# Autodesk Inventor assembly: Wall Cabinet 2 Door
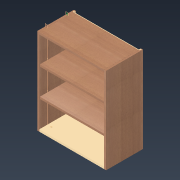
[picture p0: Inventor's stored thumbnail of the model, 180x180]
Saved by Autodesk Inventor 2022 (Build 260153000, 153)
## iProperties
Created: 2017-01-25
Part Number: Wall Cabinet 2 Door
Document SubType Name: Assembly
Designer: SvetlanaB
Author: SvetlanaB
## iProperties of the stored document MemberDocs/xAaaaqbcaAaaaaaaaAaaaqxjcCb
Created: 2017-01-25
Part Number: Wall Cabinet 2 Door
Document SubType Name: Assembly
Designer: SvetlanaB
Author: SvetlanaB
## Documents named in this file (26)
- C:\W4INV 2024 Design\iBOX LIBRARY\Kitchen\Wall Cabinets\Wall cabinet\Wall Cabinet.iam
- C:\W4INV 2022 Design\iBOX LIBRARY\Kitchen\Wall Cabinets\Wall cabinet\Right panel.ipt
- C:\W4INV 2022 Design\iBOX LIBRARY\Kitchen\Wall Cabinets\Wall cabinet\Top panel.ipt
- C:\W4INV 2022 Design\iBOX LIBRARY\Kitchen\Wall Cabinets\Wall cabinet\Bottom panel.ipt
- C:\W4INV 2022 Design\iBOX LIBRARY\Kitchen\Wall Cabinets\Wall cabinet\Left panel.ipt
- C:\W4INV 2022 Design\iBOX LIBRARY\Kitchen\Wall Cabinets\Wall cabinet\Shelf.ipt
- C:\W4INV 2022 Design\iBOX LIBRARY\Kitchen\Wall Cabinets\Wall cabinet\Back panel.ipt
- C:\W4INV 2022 Design\iBOX LIBRARY\Kitchen\Wall Cabinets\Wall cabinet\Wall Cabinet.ipt
- C:\W4INV 2022 Design\_LIBRARY\Fixed joints\Minifix joint\MINIFIX D15 v2\Minifix D15 & Dowel L34 & Cap D15 PB T18 LH.ipt
- C:\W4INV 2022 Design\_LIBRARY\Holders\Shelf holder D5\Shelf support D5 L16 with hole covers.ipt
- C:\W4INV 2022 Design\_LIBRARY\Fixed joints\Minifix joint\MINIFIX D15 v2\Minifix D15 & Dowel L34 & Cap D15 PB T18 RH.ipt
- C:\W4INV 2021 Design\LIBRARY\Fixed joints\Minifix joint\MINIFIX D15 v2.ipt
- C:\W4INV 2021 Design\LIBRARY\Holders\Shelf holder D5.ipt
- C:\W4INV 2024 Design\iBOX LIBRARY\Kitchen\Wall Cabinets\Wall cabinet\Right panel.ipt
- C:\W4INV 2024 Design\iBOX LIBRARY\Kitchen\Wall Cabinets\Wall cabinet\Top panel.ipt
- C:\W4INV 2024 Design\iBOX LIBRARY\Kitchen\Wall Cabinets\Wall cabinet\Bottom panel.ipt
- C:\W4INV 2024 Design\iBOX LIBRARY\Kitchen\Wall Cabinets\Wall cabinet\Left panel.ipt
- C:\W4INV 2024 Design\iBOX LIBRARY\Kitchen\Wall Cabinets\Wall cabinet\Shelf.ipt
- C:\W4INV 2024 Design\iBOX LIBRARY\Kitchen\Wall Cabinets\Wall cabinet\Back panel.ipt
- C:\W4INV 2024 Design\iBOX LIBRARY\Kitchen\Wall Cabinets\Wall cabinet\Wall Cabinet.ipt
- C:\W4INV 2024 Design\_LIBRARY\Fixed joints\Minifix joint\MINIFIX D15 v2\Minifix D15 & Dowel L34 & Cap D15 PB T18 LH.ipt
- C:\W4INV 2024 Design\_LIBRARY\Holders\Shelf holder D5\Shelf support D5 L16 with hole covers.ipt
- C:\W4INV 2024 Design\_LIBRARY\Fixed joints\Minifix joint\MINIFIX D15 v2\Minifix D15 & Dowel L34 & Cap D15 PB T18 RH.ipt
- C:\W4INV 2023 Design\LIBRARY\Fixed joints\Minifix joint\MINIFIX D15 v2.ipt
- C:\W4INV 2023 Design\LIBRARY\Holders\Shelf holder D5.ipt
- C:\W4INV 2022 Design\iBOX LIBRARY\Kitchen\Wall Cabinets\Wall cabinet\Wall Cabinet.iam
## Components (24 placed, 10 different names)
1. @Skeleton
2. Right panel:1 — Nestled Board Plane:5, Nestled Board Plane:6, Nestled Board Plane:7, Nestled Board Plane:8, Side Board Plane:3, Side Board Plane:4
3. Top panel:1 — Pillar Board Side Plane :1, Pillar Board Side Plane :2, Pillar Board Side Plane :5, Pillar Board Side Plane :6
4. Bottom panel:1 — Pillar Board Side Plane :3, Pillar Board Side Plane :4, Pillar Board Side Plane :7, Pillar Board Side Plane :8
5. Left panel:1 — Flush:1, Flush:2, Nestled Board Plane:1, Nestled Board Plane:2, Nestled Board Plane:3, Nestled Board Plane:4, Side Board Plane:1, Side Board Plane:2
6. Back panel:1
7. Minifix D15 & Dowel L34 & Cap D15 PB T18 RH:1 — Axis Plane:1, Nestled Board Plane:1, Pillar Board Side Plane :1
8. Minifix D15 & Dowel L34 & Cap D15 PB T18 LH:2 — Axis Plane:2, Nestled Board Plane:2, Pillar Board Side Plane :2
9. Minifix D15 & Dowel L34 & Cap D15 PB T18 LH:3 — Axis Plane:3, Nestled Board Plane:3, Pillar Board Side Plane :3
10. Minifix D15 & Dowel L34 & Cap D15 PB T18 RH:4 — Axis Plane:4, Nestled Board Plane:4, Pillar Board Side Plane :4
11. Minifix D15 & Dowel L34 & Cap D15 PB T18 LH:5 — Axis Plane:5, Nestled Board Plane:5, Pillar Board Side Plane :5
12. Minifix D15 & Dowel L34 & Cap D15 PB T18 RH:6 — Axis Plane:6, Nestled Board Plane:6, Pillar Board Side Plane :6
13. Minifix D15 & Dowel L34 & Cap D15 PB T18 LH:7 — Axis Plane:7, Nestled Board Plane:7, Pillar Board Side Plane :7
14. Minifix D15 & Dowel L34 & Cap D15 PB T18 RH:8 — Axis Plane:8, Nestled Board Plane:8, Pillar Board Side Plane :8
15. Shelf:1 — Shelf Pottom Plane:3, Shelf Pottom Plane:4, Shelf Pottom Plane:1, Shelf Pottom Plane:2
16. Shelf support D5 L16 with hole covers:1 — Side Board Plane:1, Axis Plane:9, Shelf Pottom Plane:1
17. Shelf support D5 L16 with hole covers:2 — Side Board Plane:2, Axis Plane:10, Shelf Pottom Plane:2
18. Shelf support D5 L16 with hole covers:3 — Side Board Plane:3, Shelf Pottom Plane:3, Axis Plane:11
19. Shelf support D5 L16 with hole covers:4 — Side Board Plane:4, Shelf Pottom Plane:4, Axis Plane:12
20. Shelf:2
21. Shelf support D5 L16 with hole covers:5
22. Shelf support D5 L16 with hole covers:6
23. Shelf support D5 L16 with hole covers:7
24. Shelf support D5 L16 with hole covers:8
## Component patterns: (2 elements, first: Shelf:1 + Shelf support D5 L16 with hole covers:1 + Shelf support D5 L16 with hole covers:2 + Shelf support D5 L16 with hole covers:3 + Shelf support D5 L16 with hole covers:4)
## Relationships (38: Mate 28, Flush 10)
- Flush:1 (-70 mm): Left panel:1
- Flush:2 (-70 mm): Left panel:1
- Axis Plane:1 [Mate]: Minifix D15 & Dowel L34 & Cap D15 PB T18 RH:1
- Nestled Board Plane:1 [Mate]: Left panel:1 ↔ Minifix D15 & Dowel L34 & Cap D15 PB T18 RH:1
- Pillar Board Side Plane :1 [Flush] (18 mm): Top panel:1 ↔ Minifix D15 & Dowel L34 & Cap D15 PB T18 RH:1
- Axis Plane:2 [Mate]: Minifix D15 & Dowel L34 & Cap D15 PB T18 LH:2
- Nestled Board Plane:2 [Mate]: Left panel:1 ↔ Minifix D15 & Dowel L34 & Cap D15 PB T18 LH:2
- Pillar Board Side Plane :2 [Flush] (18 mm): Top panel:1 ↔ Minifix D15 & Dowel L34 & Cap D15 PB T18 LH:2
- Axis Plane:3 [Mate]: Minifix D15 & Dowel L34 & Cap D15 PB T18 LH:3
- Nestled Board Plane:3 [Mate]: Left panel:1 ↔ Minifix D15 & Dowel L34 & Cap D15 PB T18 LH:3
- Pillar Board Side Plane :3 [Flush] (18 mm): Bottom panel:1 ↔ Minifix D15 & Dowel L34 & Cap D15 PB T18 LH:3
- Axis Plane:4 [Mate]: Minifix D15 & Dowel L34 & Cap D15 PB T18 RH:4
- Nestled Board Plane:4 [Mate]: Left panel:1 ↔ Minifix D15 & Dowel L34 & Cap D15 PB T18 RH:4
- Pillar Board Side Plane :4 [Flush] (18 mm): Bottom panel:1 ↔ Minifix D15 & Dowel L34 & Cap D15 PB T18 RH:4
- Axis Plane:5 [Mate]: Minifix D15 & Dowel L34 & Cap D15 PB T18 LH:5
- Nestled Board Plane:5 [Mate]: Right panel:1 ↔ Minifix D15 & Dowel L34 & Cap D15 PB T18 LH:5
- Pillar Board Side Plane :5 [Flush] (18 mm): Top panel:1 ↔ Minifix D15 & Dowel L34 & Cap D15 PB T18 LH:5
- Axis Plane:6 [Mate]: Minifix D15 & Dowel L34 & Cap D15 PB T18 RH:6
- Nestled Board Plane:6 [Mate]: Right panel:1 ↔ Minifix D15 & Dowel L34 & Cap D15 PB T18 RH:6
- Pillar Board Side Plane :6 [Flush] (18 mm): Top panel:1 ↔ Minifix D15 & Dowel L34 & Cap D15 PB T18 RH:6
- Axis Plane:7 [Mate]: Minifix D15 & Dowel L34 & Cap D15 PB T18 LH:7
- Nestled Board Plane:7 [Mate]: Right panel:1 ↔ Minifix D15 & Dowel L34 & Cap D15 PB T18 LH:7
- Pillar Board Side Plane :7 [Flush] (18 mm): Bottom panel:1 ↔ Minifix D15 & Dowel L34 & Cap D15 PB T18 LH:7
- Axis Plane:8 [Mate]: Minifix D15 & Dowel L34 & Cap D15 PB T18 RH:8
- Nestled Board Plane:8 [Mate]: Right panel:1 ↔ Minifix D15 & Dowel L34 & Cap D15 PB T18 RH:8
- Pillar Board Side Plane :8 [Flush] (18 mm): Bottom panel:1 ↔ Minifix D15 & Dowel L34 & Cap D15 PB T18 RH:8
- Side Board Plane:1 [Mate]: Left panel:1 ↔ Shelf support D5 L16 with hole covers:1
- Axis Plane:9 [Mate]: Shelf support D5 L16 with hole covers:1
- Side Board Plane:2 [Mate]: Left panel:1 ↔ Shelf support D5 L16 with hole covers:2
- Axis Plane:10 [Mate]: Shelf support D5 L16 with hole covers:2
- Side Board Plane:3 [Mate]: Right panel:1 ↔ Shelf support D5 L16 with hole covers:3
- Shelf Pottom Plane:3 [Mate] (2.5 mm): Shelf:1 ↔ Shelf support D5 L16 with hole covers:3
- Axis Plane:11 [Mate]: Shelf support D5 L16 with hole covers:3
- Side Board Plane:4 [Mate]: Right panel:1 ↔ Shelf support D5 L16 with hole covers:4
- Shelf Pottom Plane:4 [Mate] (2.5 mm): Shelf:1 ↔ Shelf support D5 L16 with hole covers:4
- Axis Plane:12 [Mate]: Shelf support D5 L16 with hole covers:4
- Shelf Pottom Plane:1 [Mate] (2.5 mm): Shelf:1 ↔ Shelf support D5 L16 with hole covers:1
- Shelf Pottom Plane:2 [Mate] (2.5 mm): Shelf:1 ↔ Shelf support D5 L16 with hole covers:2
## Named parameters: Shelf_quantity = 2, Panel_thickness = 18 mm, Distance_between_shelfs = 226 mm
